# Autodesk Inventor assembly: X-Gantry Assembly for 4040 V3
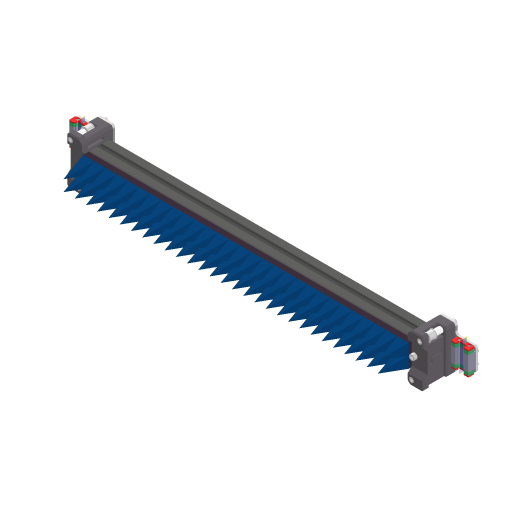
[picture p0: Inventor's stored thumbnail of the model, 512x512]
Saved by Autodesk Inventor 2023.2 (Build 272271000, 271)
## iProperties
Created: 2023-11-20
Part Number: X-Gantry Assembly for 4040 V3
Document SubType Name: Assembly
Designer: Nils Bade
Author: Nils Bade
## Documents named in this file (6)
- C:\Users\nilsb\Documents\Inventor\Projektarbeit-Bade\RatRig_Bade\X-Gantry Assembly for 4040 V3.iam
- C:\Users\nilsb\Documents\Inventor\Projektarbeit-Bade\RatRig_Bade\X-Gantry Joiner Left V4 Assembly.iam
- C:\Users\nilsb\Documents\Inventor\Projektarbeit-Bade\RatRig_Bade\X-Gantry Joiner Right V4 Assembly.iam
- C:\Users\nilsb\Documents\Inventor\Projektarbeit-Bade\ITEM\4040 Profile\ITEM T-SLOT 4040 622mm.ipt
- C:\Users\nilsb\Documents\Inventor\Projektarbeit-Bade\RatRig_modified\MGN15 Linear Rail 570mm - 4040 Assembly.iam
- C:\Users\nilsb\Documents\Inventor\Projektarbeit-Bade\Enclosure\Absorber\Absorber IHF X-Gantry.iam
## Components (5 placed, 5 different names)
1. X-Gantry Joiner Left V4 Assembly:1 [sub-assembly] — Passend:1, Passend:2, Passend:3
2. X-Gantry Joiner Right V4 Assembly:1 [sub-assembly] — Passend:4, Passend:5, Passend:6, Passend:9
3. ITEM T-SLOT 4040 622mm:1 — Passend:1, Passend:2, Passend:3, Passend:4, Passend:5, Passend:6, Fluchtend:2, Passend:10
4. MGN15 Linear Rail 570mm - 4040 Assembly:1 [sub-assembly]
5. Absorber IHF X-Gantry:1 [sub-assembly] — Fluchtend:2, Passend:9, Passend:10
## Relationships (12: Mate 10, Flush 2)
- Passend:1 [Mate]: X-Gantry Joiner Left V4 Assembly:1 ↔ ITEM T-SLOT 4040 622mm:1
- Passend:2 [Mate]: X-Gantry Joiner Left V4 Assembly:1 ↔ ITEM T-SLOT 4040 622mm:1
- Passend:3 [Mate]: X-Gantry Joiner Left V4 Assembly:1 ↔ ITEM T-SLOT 4040 622mm:1
- Passend:4 [Mate]: X-Gantry Joiner Right V4 Assembly:1 ↔ ITEM T-SLOT 4040 622mm:1
- Passend:5 [Mate]: X-Gantry Joiner Right V4 Assembly:1 ↔ ITEM T-SLOT 4040 622mm:1
- Passend:6 [Mate]: X-Gantry Joiner Right V4 Assembly:1 ↔ ITEM T-SLOT 4040 622mm:1
- [Flush]: ITEM T-SLOT 4040 622mm:1 ↔ MGN15 Linear Rail 570mm - 4040 Assembly:1
- [Mate]: ITEM T-SLOT 4040 622mm:1 ↔ MGN15 Linear Rail 570mm - 4040 Assembly:1
- [Mate]: X-Gantry Joiner Right V4 Assembly:1 ↔ MGN15 Linear Rail 570mm - 4040 Assembly:1
- Fluchtend:2 [Flush]: ITEM T-SLOT 4040 622mm:1 ↔ Absorber IHF X-Gantry:1
- Passend:9 [Mate]: X-Gantry Joiner Right V4 Assembly:1 ↔ Absorber IHF X-Gantry:1
- Passend:10 [Mate]: ITEM T-SLOT 4040 622mm:1 ↔ Absorber IHF X-Gantry:1
